# Autodesk Inventor assembly: wheelForHangingAndMovingV2
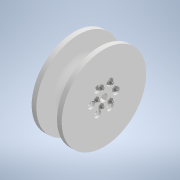
[picture p0: Inventor's stored thumbnail of the model, 180x180]
Saved by Autodesk Inventor 2020.2 (Build 242310000, 310)
## iProperties
Created: 2020-01-09
Part Number: wheelForHangingAndMovingV2
Document SubType Name: Assembly
Designer: robst
Author: robst
## Documents named in this file (3)
- C:\git\CAD-Development\robSteele\2020 Lift Mechanism\wheelForHangingAndMovingV2.iam
- C:\git\CAD-Development\robSteele\2020 Lift Mechanism\halfWheelForHangingAndMovingV2.ipt
- C:\git\CAD-Development\robSteele\2020 Lift Mechanism\wheelForHangingAndMovingV2\Design Accelerator\Bolted Connection1.iam
## Components (3 placed, 2 different names)
1. halfWheelForHangingAndMovingV2:1 — Mate:1, Mate:2, Mate:3
2. halfWheelForHangingAndMovingV2:2 — Mate:1, Mate:2, Mate:3, Mate:4, Mate:5
3. Bolted Connection:1 [sub-assembly] — Mate:4, Mate:5
## Relationships (5: Mate 5)
- Mate:1: halfWheelForHangingAndMovingV2:1 ↔ halfWheelForHangingAndMovingV2:2
- Mate:2: halfWheelForHangingAndMovingV2:1 ↔ halfWheelForHangingAndMovingV2:2
- Mate:3: halfWheelForHangingAndMovingV2:1 ↔ halfWheelForHangingAndMovingV2:2
- Mate:4: halfWheelForHangingAndMovingV2:2 ↔ Bolted Connection:1
- Mate:5: halfWheelForHangingAndMovingV2:2 ↔ Bolted Connection:1
